# Autodesk Inventor assembly: Start_Cell
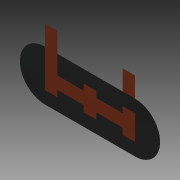
[picture p0: Inventor's stored thumbnail of the model, 180x180]
Saved by Autodesk Inventor 2014 SP1 (Build 180222100, 222)
## iProperties
Created: 2014-01-13
Part Number: Start_Cell
Document SubType Name: Assembly
Designer: tuleu
Author: tuleu
## Documents named in this file (3)
- C:\Users\tuleu\Documents\giant-snes-gamepad\cad\Start_Cell.iam
- C:\Users\tuleu\Documents\giant-snes-gamepad\cad\Start_Velostat.ipt
- C:\Users\tuleu\Documents\giant-snes-gamepad\cad\Start_Copper.ipt
## Components (3 placed, 2 different names)
1. Start_Velostat:1 — Mate:1, Mate:2, Mate:3, Mate:4, Mate:5, Mate:6
2. Start_Copper:1 — Mate:1, Mate:2, Mate:3
3. Start_Copper:2 — Mate:4, Mate:5, Mate:6
## Relationships (6: Mate 6)
- Mate:1: Start_Velostat:1 ↔ Start_Copper:1
- Mate:2: Start_Velostat:1 ↔ Start_Copper:1
- Mate:3: Start_Velostat:1 ↔ Start_Copper:1
- Mate:4: Start_Velostat:1 ↔ Start_Copper:2
- Mate:5: Start_Velostat:1 ↔ Start_Copper:2
- Mate:6: Start_Velostat:1 ↔ Start_Copper:2
